# Autodesk Inventor assembly: A2017_T4_09
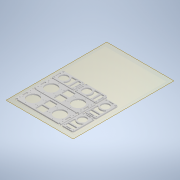
[picture p0: Inventor's stored thumbnail of the model, 180x180]
Saved by Autodesk Inventor 2020 (Build 240168000, 168)
## iProperties
Created: 2021-08-27
Part Number: A2017_T4_09
Document SubType Name: Assembly
Designer: Masato
Author: Masato
## Documents named in this file (4)
- C:\Inventor\SUSTAINA-OP\Cam\A2017_T4_09.iam
- C:\Inventor\SUSTAINA-OP\Cam\DisposableBoard.ipt
- C:\Inventor\SUSTAINA-OP\UpperBody\Trunk\Trunk_waisit_frame.ipt
- C:\Inventor\SUSTAINA-OP\UpperBody\Trunk\Trunk_neck_frame.ipt
## Components (7 placed, 3 different names)
1. DisposableBoard:1 — メイト:2, メイト:1, フラッシュ:1, フラッシュ:2, メイト:4, メイト:5, フラッシュ:3, フラッシュ:4, フラッシュ:5, メイト:7, メイト:8, メイト:9, メイト:10
2. Trunk_waisit_frame:1 — メイト:4, フラッシュ:3, フラッシュ:4, メイト:6, フラッシュ:6, フラッシュ:8, メイト:13
3. Trunk_waisit_frame:2 — メイト:5, メイト:6, フラッシュ:5, メイト:11
4. Trunk_neck_frame:1 — メイト:7, フラッシュ:8, メイト:13, メイト:14, フラッシュ:9
5. Trunk_neck_frame:2 — メイト:8, メイト:14, フラッシュ:9
6. Trunk_neck_frame:3 — メイト:10, メイト:11, フラッシュ:6, メイト:12, フラッシュ:7
7. Trunk_neck_frame:4 — メイト:9, メイト:12, フラッシュ:7
## Relationships (22: Mate 13, Flush 9)
- メイト:2 [Mate]: DisposableBoard:1
- メイト:1 [Mate]: DisposableBoard:1
- フラッシュ:1 [Flush]: DisposableBoard:1
- フラッシュ:2 [Flush]: DisposableBoard:1
- メイト:4 [Mate]: DisposableBoard:1 ↔ Trunk_waisit_frame:1
- メイト:5 [Mate]: DisposableBoard:1 ↔ Trunk_waisit_frame:2
- フラッシュ:3 [Flush] (2 mm): DisposableBoard:1 ↔ Trunk_waisit_frame:1
- フラッシュ:4 [Flush] (2 mm): DisposableBoard:1 ↔ Trunk_waisit_frame:1
- メイト:6 [Mate] (2.5 mm): Trunk_waisit_frame:1 ↔ Trunk_waisit_frame:2
- フラッシュ:5 [Flush] (2 mm): DisposableBoard:1 ↔ Trunk_waisit_frame:2
- メイト:7 [Mate]: DisposableBoard:1 ↔ Trunk_neck_frame:1
- メイト:8 [Mate]: DisposableBoard:1 ↔ Trunk_neck_frame:2
- メイト:9 [Mate]: DisposableBoard:1 ↔ Trunk_neck_frame:4
- メイト:10 [Mate]: DisposableBoard:1 ↔ Trunk_neck_frame:3
- メイト:11 [Mate] (2.5 mm): Trunk_waisit_frame:2 ↔ Trunk_neck_frame:3
- フラッシュ:6 [Flush]: Trunk_waisit_frame:1 ↔ Trunk_neck_frame:3
- メイト:12 [Mate] (2.5 mm): Trunk_neck_frame:3 ↔ Trunk_neck_frame:4
- フラッシュ:7 [Flush]: Trunk_neck_frame:3 ↔ Trunk_neck_frame:4
- フラッシュ:8 [Flush]: Trunk_waisit_frame:1 ↔ Trunk_neck_frame:1
- メイト:13 [Mate] (2.5 mm): Trunk_waisit_frame:1 ↔ Trunk_neck_frame:1
- メイト:14 [Mate] (2.5 mm): Trunk_neck_frame:1 ↔ Trunk_neck_frame:2
- フラッシュ:9 [Flush]: Trunk_neck_frame:1 ↔ Trunk_neck_frame:2
